# Autodesk Inventor assembly: MultiRig
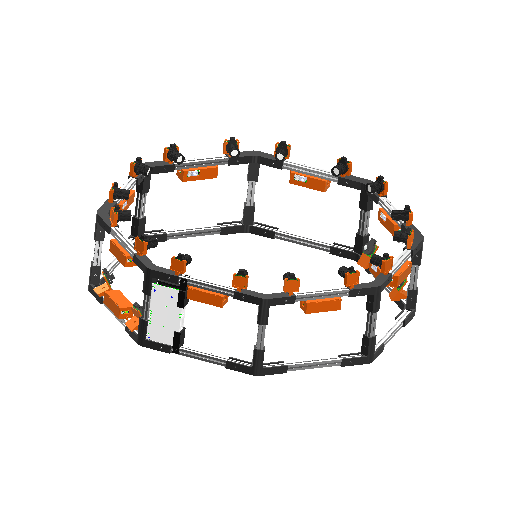
[picture p0: Inventor's stored thumbnail of the model, 512x512]
Saved by Autodesk Inventor 2025.2 (Build 292293000, 293)
## iProperties
Created: 2025-03-12
Part Number: MultiRig
Document SubType Name: Assembly
Designer: rolan
Author: rolan
## Documents named in this file (6)
- C:\Users\rolan\Documents\PhD\Inventor\Assembly\MultiRig.iam
- C:\Users\rolan\Documents\PhD\Inventor\Assembly\SubAssembly.iam
- C:\Users\rolan\Documents\PhD\Inventor\Assembly\PowerSupply.iam
- C:\Users\rolan\Documents\PhD\Inventor\Assembly\StereoPiM12.iam
- C:\Users\rolan\Documents\PhD\Inventor\Assembly\M12Cam.iam
- C:\Users\rolan\Documents\PhD\Inventor\Assembly\M12CamMirror.iam
## Components (15 placed, 5 different names)
1. SubAssembly:1 [sub-assembly] — Mate:1, Mate:2, Mate:3
2. SubAssembly:2 [sub-assembly] — Mate:1, Mate:2, Mate:3, Mate:4, Mate:5, Mate:6
3. SubAssembly:3 [sub-assembly] — Mate:4, Mate:5, Mate:6, Mate:7, Mate:8, Mate:9, Flush:43, Mate:43, Mate:44, Mate:45, Mate:46, Mate:47, Mate:48
4. SubAssembly:4 [sub-assembly] — Mate:7, Mate:8, Mate:9, Mate:10, Mate:11, Mate:12, Mate:56, Mate:57, Mate:58
5. SubAssembly:5 [sub-assembly] — Mate:10, Mate:11, Mate:12, Mate:13, Mate:14, Mate:15
6. SubAssembly:6 [sub-assembly] — Mate:13, Mate:14, Mate:15, Mate:16, Mate:17, Mate:18, Mate:22, Mate:23
7. SubAssembly:7 [sub-assembly] — Mate:16, Mate:17, Mate:18, Mate:19, Mate:20, Mate:21, Flush:44, Mate:41, Mate:52
8. SubAssembly:8 [sub-assembly] — Mate:19, Mate:20, Mate:21, Mate:49, Mate:50, Mate:51, Mate:53, Mate:54, Mate:55
9. PowerSupply:1 [sub-assembly] — Mate:22, Mate:23
10. StereoPiM12:1 [sub-assembly] — Flush:44, Mate:41
11. StereoPiM12:2 [sub-assembly] — Flush:43, Mate:43
12. M12Cam:1 [sub-assembly] — Mate:44, Mate:45, Mate:46, Mate:47, Mate:48
13. M12Cam:2 [sub-assembly] — Mate:49, Mate:50, Mate:51, Mate:52
14. M12CamMirror:1 [sub-assembly] — Mate:53, Mate:54, Mate:55
15. M12CamMirror:2 [sub-assembly] — Mate:56, Mate:57, Mate:58
## Relationships (42: Mate 40, Flush 2)
- Mate:1: SubAssembly:1 ↔ SubAssembly:2
- Mate:2: SubAssembly:1 ↔ SubAssembly:2
- Mate:3: SubAssembly:1 ↔ SubAssembly:2
- Mate:4: SubAssembly:2 ↔ SubAssembly:3
- Mate:5: SubAssembly:2 ↔ SubAssembly:3
- Mate:6: SubAssembly:2 ↔ SubAssembly:3
- Mate:7: SubAssembly:3 ↔ SubAssembly:4
- Mate:8: SubAssembly:3 ↔ SubAssembly:4
- Mate:9: SubAssembly:3 ↔ SubAssembly:4
- Mate:10: SubAssembly:4 ↔ SubAssembly:5
- Mate:11: SubAssembly:4 ↔ SubAssembly:5
- Mate:12: SubAssembly:4 ↔ SubAssembly:5
- Mate:13: SubAssembly:5 ↔ SubAssembly:6
- Mate:14: SubAssembly:5 ↔ SubAssembly:6
- Mate:15: SubAssembly:5 ↔ SubAssembly:6
- Mate:16: SubAssembly:6 ↔ SubAssembly:7
- Mate:17: SubAssembly:6 ↔ SubAssembly:7
- Mate:18: SubAssembly:6 ↔ SubAssembly:7
- Mate:19: SubAssembly:7 ↔ SubAssembly:8
- Mate:20: SubAssembly:7 ↔ SubAssembly:8
- Mate:21: SubAssembly:7 ↔ SubAssembly:8
- Mate:22: SubAssembly:6 ↔ PowerSupply:1
- Mate:23: SubAssembly:6 ↔ PowerSupply:1
- Flush:44: SubAssembly:7 ↔ StereoPiM12:1
- Mate:41: SubAssembly:7 ↔ StereoPiM12:1
- Flush:43: SubAssembly:3 ↔ StereoPiM12:2
- Mate:43: SubAssembly:3 ↔ StereoPiM12:2
- Mate:44: SubAssembly:3 ↔ M12Cam:1
- Mate:45: SubAssembly:3 ↔ M12Cam:1
- Mate:46: SubAssembly:3 ↔ M12Cam:1
- Mate:47: SubAssembly:3 ↔ M12Cam:1
- Mate:48: SubAssembly:3 ↔ M12Cam:1
- Mate:49: SubAssembly:8 ↔ M12Cam:2
- Mate:50: SubAssembly:8 ↔ M12Cam:2
- Mate:51: SubAssembly:8 ↔ M12Cam:2
- Mate:52: SubAssembly:7 ↔ M12Cam:2
- Mate:53: SubAssembly:8 ↔ M12CamMirror:1
- Mate:54: SubAssembly:8 ↔ M12CamMirror:1
- Mate:55: SubAssembly:8 ↔ M12CamMirror:1
- Mate:56: SubAssembly:4 ↔ M12CamMirror:2
- Mate:57: SubAssembly:4 ↔ M12CamMirror:2
- Mate:58: SubAssembly:4 ↔ M12CamMirror:2
